# Autodesk Inventor assembly: Top Roller
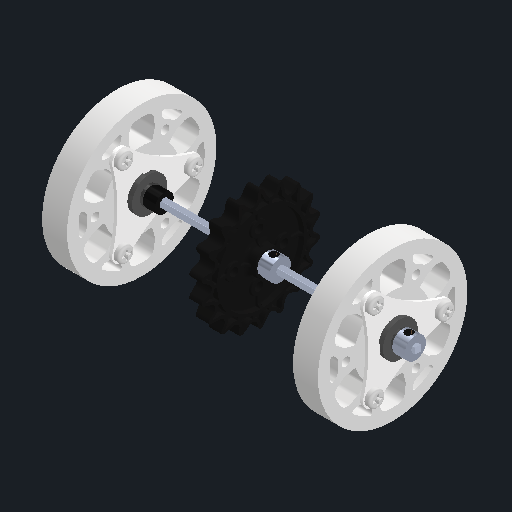
[picture p0: Inventor's stored thumbnail of the model, 512x512]
Saved by Autodesk Inventor 2025 (Build 290162000, 162)
## iProperties
Created: 2024-12-29
Part Number: Top Roller
Document SubType Name: Assembly
Designer: Averey Ku
Author: Averey Ku
## Documents named in this file (10)
- D:\VEX\High Stakes\CAD\V4\Conveyer\Top Roller.iam
- D:\VEX\High Stakes\CAD\ROBOPROS-CAD-Inventor\Quick Assemblies\3.000 30A .500 With Adapters.iam
- D:\VEX\High Stakes\CAD\ROBOPROS-CAD-Inventor\Motion\Insert Square.ipt
- D:\VEX\High Stakes\CAD\ROBOPROS-CAD-Inventor\Motion\Spacers\Spacer Nylon .375 OD\NSpacer .375 OD x .250.ipt
- D:\VEX\High Stakes\CAD\ROBOPROS-CAD-Inventor\Motion\Spacers\Spacer Nylon .375 OD.ipt
- D:\VEX\High Stakes\CAD\ROBOPROS-CAD-Inventor\Motion\Shaft LS\Shaft Collar ipts\Shaft Collar Set Screw.ipt
- D:\VEX\High Stakes\CAD\ROBOPROS-CAD-Inventor\Motion\Sprockets\9P Sprocket\9P 18T Sprocket, Square.iam
- D:\VEX\High Stakes\CAD\ROBOPROS-CAD-Inventor\Motion\Sprockets\9P Sprocket.iam
- D:\VEX\High Stakes\CAD\ROBOPROS-CAD-Inventor\Motion\Shaft LS\Shaft LS\Shaft LS 6.5.ipt
- D:\VEX\High Stakes\CAD\ROBOPROS-CAD-Inventor\Motion\Shaft LS\Shaft LS.ipt
## Components (14 placed, 6 different names)
1. 3.000 30A .500 With Adapters:1 [sub-assembly] — Insert:1, Insert:2
2. Insert Square:1 — Insert:2, Mate:1, Mate:2, Insert:3, Flush:1
3. Insert Square:2 — Insert:1, Insert:4
4. NSpacer .375 OD x .250:1 — Insert:3, Insert:9
5. Shaft Collar Set Screw:1 — Insert:4, Insert:10
6. 3.000 30A .500 With Adapters:2 [sub-assembly] — Insert:5, Insert:6
7. Insert Square:3 — Mate:4, Mate:5, Insert:5, Insert:7, Mate:3
8. Insert Square:4 — Insert:6, Insert:8
9. NSpacer .375 OD x .250:2 — Insert:7
10. Shaft Collar Set Screw:2 — Insert:8
11. 9P 18T Sprocket, Square:1 [sub-assembly] — Insert:9, Insert:11, Insert:12
12. Shaft LS 6.5:1 — Insert:10
13. Shaft Collar Set Screw:3 — Insert:11
14. Shaft Collar Set Screw:4 — Insert:12
## Relationships (18: Insert 12, Mate 5, Flush 1)
- Insert:1: 3.000 30A .500 With Adapters:1 ↔ Insert Square:2
- Insert:2: 3.000 30A .500 With Adapters:1 ↔ Insert Square:1
- Flush:1 (52.3875 mm): Insert Square:1
- Mate:1: Insert Square:1
- Mate:2: Insert Square:1
- Insert:3: Insert Square:1 ↔ NSpacer .375 OD x .250:1
- Insert:4: Insert Square:2 ↔ Shaft Collar Set Screw:1
- Mate:3 (52.3875 mm): Insert Square:3
- Mate:4: Insert Square:3
- Mate:5: Insert Square:3
- Insert:5: 3.000 30A .500 With Adapters:2 ↔ Insert Square:3
- Insert:6: 3.000 30A .500 With Adapters:2 ↔ Insert Square:4
- Insert:7: Insert Square:3 ↔ NSpacer .375 OD x .250:2
- Insert:8: Insert Square:4 ↔ Shaft Collar Set Screw:2
- Insert:9 (39.37 mm): NSpacer .375 OD x .250:1 ↔ 9P 18T Sprocket, Square:1
- Insert:10: Shaft Collar Set Screw:1 ↔ Shaft LS 6.5:1
- Insert:11: 9P 18T Sprocket, Square:1 ↔ Shaft Collar Set Screw:3
- Insert:12: 9P 18T Sprocket, Square:1 ↔ Shaft Collar Set Screw:4
